# Autodesk Inventor assembly: Chain Drive
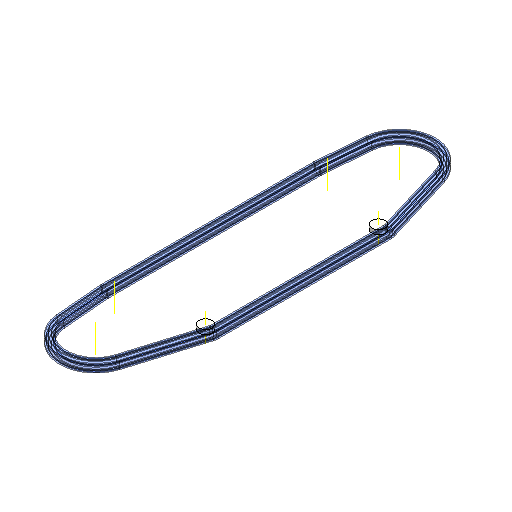
[picture p0: Inventor's stored thumbnail of the model, 512x512]
Saved by Autodesk Inventor 2025 (Build 290162000, 162)
## iProperties
ClientObjectVersion: 1
Created: 2024-07-22
Part Number: Chain Drive
Document SubType Name: Assembly
Designer: seene
Author: seene
## Documents named in this file (4)
- C:\Users\seene\Desktop\Stony Brook\SBRT\RCR_Dexter\Drive\RCR_drive\Design Accelerator\Chain Drive2.iam
- C:\Users\seene\Desktop\Stony Brook\SBRT\RCR_Dexter\Drive\RCR_drive\Design Accelerator\Roller Chain2.ipt
- C:\Users\seene\Desktop\Stony Brook\SBRT\RCR_Dexter\Drive\RCR_drive\Design Accelerator\Flat Idler11.ipt
- C:\Users\seene\Desktop\Stony Brook\SBRT\RCR_Dexter\Drive\RCR_drive\Design Accelerator\Flat Idler21.ipt
## Components (3 placed, 3 different names)
1. Roller Chain:1 — Flush:1, Mate:1, Flush:2, Mate:2
2. Flat Idler1:1 — Flush:1, Mate:1
3. Flat Idler2:1 — Flush:2, Mate:2
## Relationships (4: Flush 2, Mate 2)
- Flush:1: Roller Chain:1 ↔ Flat Idler1:1
- Mate:1: Roller Chain:1 ↔ Flat Idler1:1
- Flush:2: Roller Chain:1 ↔ Flat Idler2:1
- Mate:2: Roller Chain:1 ↔ Flat Idler2:1
